# Autodesk Inventor assembly: Red+Black License plate with numbers
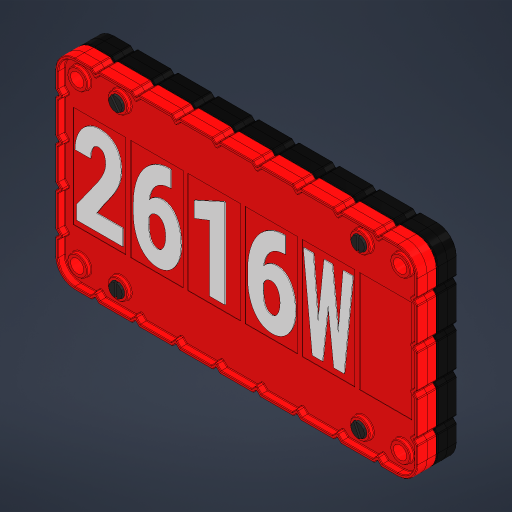
[picture p0: Inventor's stored thumbnail of the model, 512x512]
Saved by Autodesk Inventor 2023.2 (Build 272271030, 271C)
## iProperties
Created: 2023-05-28
Part Number: Red+Black License plate with numbers
Document SubType Name: Assembly
Designer: Main Account
Author: Main Account
## Documents named in this file (6)
- C:\Users\Main Account\InventorProjects\VEX\Custom Library\Red+Black License plate with numbers.iam
- C:\Users\Main Account\InventorProjects\VEX\Custom Library\Black License Plate.ipt
- C:\Users\Main Account\InventorProjects\VEX\Library Backup\Library 1.4\Miscellaneous\Red License Plate.ipt
- C:\Users\Main Account\InventorProjects\VEX\Custom Library\License Plate Numbers.ipt
- License Plate Numbers.ipt
- C:\Users\Main Account\InventorProjects\VEX\Library Backup\Library 1.4\Structure\Hardware\VEX IQ Pin.ipt
## Components (7 placed, 4 different names)
1. Black License Plate:1 — Insert:1, Insert:2, Insert:3, Insert:4
2. Red License Plate:1 — Insert:5, Insert:6, Mate:1, Mate:2, Mate:3
3. License Plate Numbers:1 — Mate:1, Mate:2, Mate:3
4. VEX IQ Pin:1 — Insert:1, Insert:6
5. VEX IQ Pin:2 — Insert:2
6. VEX IQ Pin:3 — Insert:4, Insert:5
7. VEX IQ Pin:4 — Insert:3
## Relationships (9: Insert 6, Mate 3)
- Insert:1: Black License Plate:1 ↔ VEX IQ Pin:1
- Insert:2: Black License Plate:1 ↔ VEX IQ Pin:2
- Insert:3: Black License Plate:1 ↔ VEX IQ Pin:4
- Insert:4: Black License Plate:1 ↔ VEX IQ Pin:3
- Insert:5: Red License Plate:1 ↔ VEX IQ Pin:3
- Insert:6: Red License Plate:1 ↔ VEX IQ Pin:1
- Mate:1: Red License Plate:1 ↔ License Plate Numbers:1
- Mate:2: Red License Plate:1 ↔ License Plate Numbers:1
- Mate:3: Red License Plate:1 ↔ License Plate Numbers:1
